# Autodesk Inventor assembly: 100-10-FRAME-DIFFERENTIAL-01
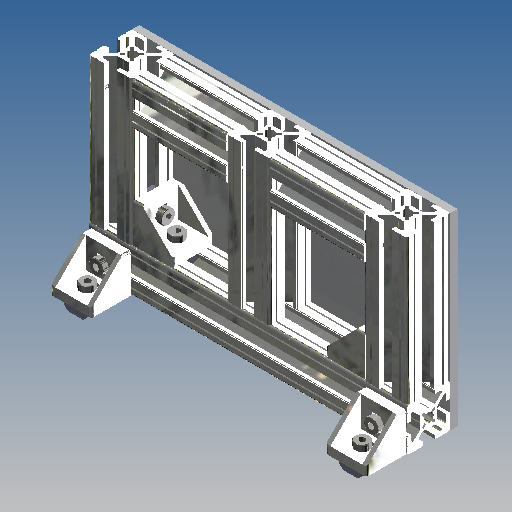
[picture p0: Inventor's stored thumbnail of the model, 512x512]
Saved by Autodesk Inventor 2018.2 (Build 222227000, 227)
## iProperties
Manager: feesmrt
Company: FRANCOR
Part Number: 100-10-FRAME-DIFFERENTIAL-01
Project: Rescue Robot
Cost Center: -
Material: Generisch
Document SubType Name: Assembly
Designer: feesmrt
Engineer: feesmrt
Authority: feesmrt
Description: Differential Profile Setup
Stock Number: 100-10-FRAME-DIFFERENTIAL-01
Subject: Rescue Robot
Author: feesmrt
Revision Number: 1
Title: Differential Profile Setup
## Documents named in this file (10)
- C:\Users\feesmrt\Documents\FRANC0R\CAD\02-Rocker-Bogie-Robot\100-CHASSIS\10-FRAME\100-10-FRAME-DIFFERENTIAL-01.iam
- C:\Users\feesmrt\Documents\FRANC0R\CAD\02-Rocker-Bogie-Robot\100-CHASSIS\10-FRAME\100-10-FRAME-PROFILE-DIFFERENTIAL-H.ipt
- C:\Users\feesmrt\Documents\FRANC0R\CAD\02-Rocker-Bogie-Robot\100-CHASSIS\10-FRAME\100-10-FRAME-PROFILE-DIFFERENTIAL-W.ipt
- C:\Users\feesmrt\Documents\FRANC0R\CAD\02-Rocker-Bogie-Robot\100-CHASSIS\10-FRAME\100-10-FRAME-DIFFERENTIAL-REINF-01.iam
- C:\Users\feesmrt\Documents\FRANC0R\CAD\02-Rocker-Bogie-Robot\900-COMPONENTS\900-80-WASHERS\900-80-WASHERS-DIN9021-M8.ipt
- C:\Users\feesmrt\Documents\FRANC0R\CAD\02-Rocker-Bogie-Robot\900-COMPONENTS\900-40-SCREWS\900-40-SCREWS-DIN7984_M8x45.ipt
- C:\Users\feesmrt\Documents\FRANC0R\CAD\02-Rocker-Bogie-Robot\900-COMPONENTS\900-50-PROFILES\900-50-PROFILES-ANGLE-CONN-30x30-01.iam
- C:\Users\feesmrt\Documents\FRANC0R\CAD\02-Rocker-Bogie-Robot\100-CHASSIS\10-FRAME\100-10-FRAME-PROFILE-WIDTH-02.ipt
- C:\Users\feesmrt\Documents\FRANC0R\CAD\02-Rocker-Bogie-Robot\900-COMPONENTS\900-50-PROFILES\900-50-PROFILES-ANGLE-CONN-30x30-02.iam
- C:\Users\feesmrt\Documents\FRANC0R\CAD\02-Rocker-Bogie-Robot\900-COMPONENTS\900-40-SCREWS\900-40-SCREWS-ISO7380_M8x16.ipt
## Components (15 placed, 9 different names)
1. 100-10-FRAME-PROFILE-DIFFERENTIAL-H:1 — Passend:1, Passend:2, Fluchtend:1, Passend:3, Passend:4, Fluchtend:2, Fluchtend:3, Fluchtend:4, Fluchtend:5, Passend:26, Passend:29
2. 100-10-FRAME-PROFILE-DIFFERENTIAL-H:2 — Passend:5, Passend:6, Fluchtend:6, Passend:40, Passend:41, Passend:47
3. 100-10-FRAME-PROFILE-DIFFERENTIAL-H:3 — Passend:7, Passend:8, Fluchtend:7, Passend:27, Passend:43, Passend:44, Passend:49
4. 100-10-FRAME-PROFILE-DIFFERENTIAL-W:1 — Passend:3, Fluchtend:3, Fluchtend:4, Passend:5, Passend:6, Fluchtend:6, Passend:46
5. 100-10-FRAME-PROFILE-DIFFERENTIAL-W:2 — Passend:4, Fluchtend:2, Fluchtend:5, Passend:7, Passend:8, Fluchtend:7, Passend:28, Passend:48
6. 100-10-FRAME-PROFILE-WIDTH-02:1 — Passend:26, Passend:30, Passend:31, Fluchtend:8, Passend:32, Passend:33, Passend:36, Passend:37, Passend:38, Passend:39, Passend:42, Passend:45, Fluchtend:9, Fluchtend:10
7. 100-10-FRAME-DIFFERENTIAL-REINF-01:1 [sub-assembly] — Passend:27, Passend:28, Passend:29, Passend:30, Passend:31, Fluchtend:8
8. 900-80-WASHERS-DIN9021-M8:3 — Passend:32, Passend:33, Passend:34, Passend:35
9. 900-40-SCREWS-DIN7984_M8x45:3 — Passend:34, Passend:35
10. 900-50-PROFILES-ANGLE-CONN-30x30-02:1 [sub-assembly] — Passend:36, Passend:39, Fluchtend:9
11. 900-50-PROFILES-ANGLE-CONN-30x30-02:2 [sub-assembly] — Passend:37, Passend:38, Fluchtend:10
12. 900-50-PROFILES-ANGLE-CONN-30x30-01:3 [sub-assembly] — Passend:40, Passend:41, Passend:42
13. 900-50-PROFILES-ANGLE-CONN-30x30-01:4 [sub-assembly] — Passend:43, Passend:44, Passend:45
14. 900-40-SCREWS-ISO7380_M8x16:1 — Passend:46, Passend:47
15. 900-40-SCREWS-ISO7380_M8x16:2 — Passend:48, Passend:49
## Relationships (42: Mate 32, Flush 10)
- Passend:1 [Mate]: 100-10-FRAME-PROFILE-DIFFERENTIAL-H:1
- Passend:2 [Mate]: 100-10-FRAME-PROFILE-DIFFERENTIAL-H:1
- Fluchtend:1 [Flush]: 100-10-FRAME-PROFILE-DIFFERENTIAL-H:1
- Passend:3 [Mate]: 100-10-FRAME-PROFILE-DIFFERENTIAL-H:1 ↔ 100-10-FRAME-PROFILE-DIFFERENTIAL-W:1
- Passend:4 [Mate]: 100-10-FRAME-PROFILE-DIFFERENTIAL-H:1 ↔ 100-10-FRAME-PROFILE-DIFFERENTIAL-W:2
- Fluchtend:2 [Flush]: 100-10-FRAME-PROFILE-DIFFERENTIAL-H:1 ↔ 100-10-FRAME-PROFILE-DIFFERENTIAL-W:2
- Fluchtend:3 [Flush]: 100-10-FRAME-PROFILE-DIFFERENTIAL-H:1 ↔ 100-10-FRAME-PROFILE-DIFFERENTIAL-W:1
- Fluchtend:4 [Flush]: 100-10-FRAME-PROFILE-DIFFERENTIAL-H:1 ↔ 100-10-FRAME-PROFILE-DIFFERENTIAL-W:1
- Fluchtend:5 [Flush]: 100-10-FRAME-PROFILE-DIFFERENTIAL-H:1 ↔ 100-10-FRAME-PROFILE-DIFFERENTIAL-W:2
- Passend:5 [Mate]: 100-10-FRAME-PROFILE-DIFFERENTIAL-H:2 ↔ 100-10-FRAME-PROFILE-DIFFERENTIAL-W:1
- Passend:6 [Mate]: 100-10-FRAME-PROFILE-DIFFERENTIAL-H:2 ↔ 100-10-FRAME-PROFILE-DIFFERENTIAL-W:1
- Fluchtend:6 [Flush]: 100-10-FRAME-PROFILE-DIFFERENTIAL-H:2 ↔ 100-10-FRAME-PROFILE-DIFFERENTIAL-W:1
- Passend:7 [Mate]: 100-10-FRAME-PROFILE-DIFFERENTIAL-H:3 ↔ 100-10-FRAME-PROFILE-DIFFERENTIAL-W:2
- Passend:8 [Mate]: 100-10-FRAME-PROFILE-DIFFERENTIAL-H:3 ↔ 100-10-FRAME-PROFILE-DIFFERENTIAL-W:2
- Fluchtend:7 [Flush]: 100-10-FRAME-PROFILE-DIFFERENTIAL-H:3 ↔ 100-10-FRAME-PROFILE-DIFFERENTIAL-W:2
- Passend:26 [Mate]: 100-10-FRAME-PROFILE-DIFFERENTIAL-H:1 ↔ 100-10-FRAME-PROFILE-WIDTH-02:1
- Passend:27 [Mate]: 100-10-FRAME-PROFILE-DIFFERENTIAL-H:3 ↔ 100-10-FRAME-DIFFERENTIAL-REINF-01:1
- Passend:28 [Mate]: 100-10-FRAME-PROFILE-DIFFERENTIAL-W:2 ↔ 100-10-FRAME-DIFFERENTIAL-REINF-01:1
- Passend:29 [Mate]: 100-10-FRAME-PROFILE-DIFFERENTIAL-H:1 ↔ 100-10-FRAME-DIFFERENTIAL-REINF-01:1
- Passend:30 [Mate]: 100-10-FRAME-PROFILE-WIDTH-02:1 ↔ 100-10-FRAME-DIFFERENTIAL-REINF-01:1
- Passend:31 [Mate]: 100-10-FRAME-PROFILE-WIDTH-02:1 ↔ 100-10-FRAME-DIFFERENTIAL-REINF-01:1
- Fluchtend:8 [Flush]: 100-10-FRAME-PROFILE-WIDTH-02:1 ↔ 100-10-FRAME-DIFFERENTIAL-REINF-01:1
- Passend:32 [Mate]: 100-10-FRAME-PROFILE-WIDTH-02:1 ↔ 900-80-WASHERS-DIN9021-M8:3
- Passend:33 [Mate]: 100-10-FRAME-PROFILE-WIDTH-02:1 ↔ 900-80-WASHERS-DIN9021-M8:3
- Passend:34 [Mate]: 900-80-WASHERS-DIN9021-M8:3 ↔ 900-40-SCREWS-DIN7984_M8x45:3
- Passend:35 [Mate]: 900-80-WASHERS-DIN9021-M8:3 ↔ 900-40-SCREWS-DIN7984_M8x45:3
- Passend:36 [Mate]: 100-10-FRAME-PROFILE-WIDTH-02:1 ↔ 900-50-PROFILES-ANGLE-CONN-30x30-02:1
- Passend:37 [Mate]: 100-10-FRAME-PROFILE-WIDTH-02:1 ↔ 900-50-PROFILES-ANGLE-CONN-30x30-02:2
- Passend:38 [Mate]: 100-10-FRAME-PROFILE-WIDTH-02:1 ↔ 900-50-PROFILES-ANGLE-CONN-30x30-02:2
- Passend:39 [Mate]: 100-10-FRAME-PROFILE-WIDTH-02:1 ↔ 900-50-PROFILES-ANGLE-CONN-30x30-02:1
- Passend:40 [Mate]: 100-10-FRAME-PROFILE-DIFFERENTIAL-H:2 ↔ 900-50-PROFILES-ANGLE-CONN-30x30-01:3
- Passend:41 [Mate]: 100-10-FRAME-PROFILE-DIFFERENTIAL-H:2 ↔ 900-50-PROFILES-ANGLE-CONN-30x30-01:3
- Passend:42 [Mate]: 100-10-FRAME-PROFILE-WIDTH-02:1 ↔ 900-50-PROFILES-ANGLE-CONN-30x30-01:3
- Passend:43 [Mate]: 100-10-FRAME-PROFILE-DIFFERENTIAL-H:3 ↔ 900-50-PROFILES-ANGLE-CONN-30x30-01:4
- Passend:44 [Mate]: 100-10-FRAME-PROFILE-DIFFERENTIAL-H:3 ↔ 900-50-PROFILES-ANGLE-CONN-30x30-01:4
- Passend:45 [Mate]: 100-10-FRAME-PROFILE-WIDTH-02:1 ↔ 900-50-PROFILES-ANGLE-CONN-30x30-01:4
- Fluchtend:9 [Flush] (1 mm): 100-10-FRAME-PROFILE-WIDTH-02:1 ↔ 900-50-PROFILES-ANGLE-CONN-30x30-02:1
- Fluchtend:10 [Flush] (1 mm): 100-10-FRAME-PROFILE-WIDTH-02:1 ↔ 900-50-PROFILES-ANGLE-CONN-30x30-02:2
- Passend:46 [Mate]: 100-10-FRAME-PROFILE-DIFFERENTIAL-W:1 ↔ 900-40-SCREWS-ISO7380_M8x16:1
- Passend:47 [Mate]: 100-10-FRAME-PROFILE-DIFFERENTIAL-H:2 ↔ 900-40-SCREWS-ISO7380_M8x16:1
- Passend:48 [Mate]: 100-10-FRAME-PROFILE-DIFFERENTIAL-W:2 ↔ 900-40-SCREWS-ISO7380_M8x16:2
- Passend:49 [Mate]: 100-10-FRAME-PROFILE-DIFFERENTIAL-H:3 ↔ 900-40-SCREWS-ISO7380_M8x16:2
